# Autodesk Inventor assembly: Hoja oculta
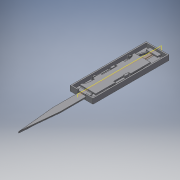
[picture p0: Inventor's stored thumbnail of the model, 180x180]
Saved by Autodesk Inventor 2016 (Build 200138000, 138)
## iProperties
Created: 2015-08-31
Part Number: Hoja oculta
Document SubType Name: Assembly
Designer: amatiasq
Author: amatiasq
## Documents named in this file (7)
- C:\Users\amatiasq\Documents\GitHub\3D\Hoja Oculta\Hoja oculta.iam
- C:\Users\amatiasq\Documents\GitHub\3D\Hoja Oculta\Base.ipt
- C:\Users\amatiasq\Documents\GitHub\3D\Hoja Oculta\Hoja.ipt
- C:\Users\amatiasq\Documents\GitHub\3D\Hoja Oculta\Tirador.ipt
- C:\Users\amatiasq\Documents\GitHub\3D\Hoja Oculta\Deslizador.ipt
- C:\Users\amatiasq\Documents\GitHub\3D\Hoja Oculta\Traba.ipt
- C:\Users\amatiasq\Documents\GitHub\3D\Hoja Oculta\Parametros.xlsx
## Components (7 placed, 5 different names)
1. Base:1 — Hoja alto, Hoja lateral, Hoja Movimiento, Base-Tirador2, Base-Tirador1, Deslizador Altura, Deslizador Lateral, Deslizador tope cola, Deslizador tope punta, Traba2 Posicion, Traba1 Posicion, Traba2 Movimiento, Traba1 Movimiento
2. Hoja:1 — Hoja alto, Hoja lateral, Hoja Movimiento, Tirador2 Alto, Hoja-Tirador2, Tirador2 Lateral, Tirador1 Lateral, Tirador1 Alto, Hoja-Tirador1
3. Tirador:1 — Base-Tirador1, Tirador1 Lateral, Tirador1 Alto, Hoja-Tirador1, Deslizador - Tirador1
4. Tirador:2 — Base-Tirador2, Tirador2 Alto, Hoja-Tirador2, Tirador2 Lateral, Deslizador - Tirador2
5. Deslizador:1 — Deslizador Altura, Deslizador Lateral, Deslizador - Tirador2, Deslizador - Tirador1, Deslizador tope cola, Deslizador tope punta
6. Traba:1 — Traba1 Posicion, Traba1 Movimiento
7. Traba:2 — Traba2 Posicion, Traba2 Movimiento
## Relationships (21: Mate 17, Insert 2, Angle 2)
- Hoja alto [Mate] (0.3 mm): Base:1 ↔ Hoja:1
- Hoja lateral [Mate]: Base:1 ↔ Hoja:1
- Hoja Movimiento [Mate]: Base:1 ↔ Hoja:1
- Base-Tirador2 [Mate]: Base:1 ↔ Tirador:2
- Tirador2 Alto [Mate] (0.3 mm): Hoja:1 ↔ Tirador:2
- Hoja-Tirador2 [Mate]: Hoja:1 ↔ Tirador:2
- Tirador2 Lateral [Mate] (0.3 mm): Hoja:1 ↔ Tirador:2
- Base-Tirador1 [Mate]: Base:1 ↔ Tirador:1
- Tirador1 Lateral [Mate] (0.3 mm): Hoja:1 ↔ Tirador:1
- Tirador1 Alto [Mate] (0.3 mm): Hoja:1 ↔ Tirador:1
- Hoja-Tirador1 [Mate]: Hoja:1 ↔ Tirador:1
- Deslizador Altura [Mate] (0.3 mm): Base:1 ↔ Deslizador:1
- Deslizador Lateral [Mate] (0.3 mm): Base:1 ↔ Deslizador:1
- Deslizador - Tirador2 [Mate]: Tirador:2 ↔ Deslizador:1
- Deslizador - Tirador1 [Mate]: Tirador:1 ↔ Deslizador:1
- Deslizador tope cola [Mate]: Base:1 ↔ Deslizador:1
- Deslizador tope punta [Mate]: Base:1 ↔ Deslizador:1
- Traba2 Posicion [Insert]: Base:1 ↔ Traba:2
- Traba1 Posicion [Insert]: Base:1 ↔ Traba:1
- Traba2 Movimiento [Angle] (18 deg): Base:1 ↔ Traba:2
- Traba1 Movimiento [Angle] (18 deg): Base:1 ↔ Traba:1
## Named parameters: margen = 0.3 mm, base_largo = 200 mm, base_ancho = 60 mm, base_alto = 3 mm, muros_grosor = 3 mm, muros_alto = 10 mm, rail_alto = 1.5 mm, rail_grosor = 5 mm, hoja_ancho = 20 mm, hoja_largo = 200 mm, hoja_filo = 100 mm, hoja_stop_posicion = 5 mm, hoja_stop_saliente = 5 mm, hoja_stop_largo = 5 mm, hoja_alto = 3 mm, hoja_stop_biselado = 2 mm, hoja_filo_biselado = 0.5 mm, hoja_cola_biselado = 1 mm, hoja_ancho_total = 30 mm, deslizador_soporte_ancho = 5 mm, deslizador_soporte_largo = 90 mm, deslizador_tope_alto = 5 mm, deslizador_soporte_alto = 4 mm, deslizador_tope_largo = 10 mm, deslizador_alto = 3 mm, tirador_agarre_largo = 3 mm, tirador_largo = 10 mm, movimiento_hoja = 200 mm, movimiento_deslizador = 30 mm, deslizador_saliente_largo = 20 mm, deslizador_saliente = 5 mm, deslizador_largo = 144 mm, deslizador_interruptor_largo = 5 mm, deslizador_interruptor_angulo = 20 mm, deslizador_interruptor_ancho = 7 mm, deslizador_ancho = 30 mm, movimiento_tirador = 30 mm, traba_ancho = 3 mm, traba_diametro_perforacion = 2 mm, traba_diametro = 5 mm, traba_top_largo = 5 mm, traba_largo = 39 mm, traba_top_alto = 3 mm, traba_alto = 4 mm, base_distancia_agujeros = 40 mm, base_separacion_agujeros = 4 mm, base_agujeros_distancia = 50 mm, base_agujeros_separacion = 3.5 mm, base_agujeros_diametro = 2 mm
